# Autodesk Inventor assembly: CarAssembly mk2
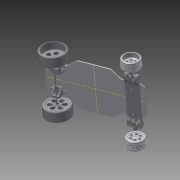
[picture p0: Inventor's stored thumbnail of the model, 180x180]
Saved by Autodesk Inventor 2015 (Build 190159000, 159)
## iProperties
Created: 2014-11-06
Part Number: CarAssembly mk2
Document SubType Name: Assembly
Designer: ah14592
Author: ah14592
## Documents named in this file (10)
- C:\Users\ah14592\Desktop\Inventor\Assembly\CarAssembly mk2.iam
- C:\Users\ah14592\Desktop\Inventor\Steering\Steering Rod\mk1.ipt
- C:\Users\ah14592\Desktop\Inventor\Steering\Steering T\Part3.ipt
- C:\Users\ah14592\Desktop\Inventor\Steering\T Connector Rod\Part1.ipt
- C:\Users\ah14592\Desktop\Inventor\Wheels\Front Wheels\Wheels1.ipt
- C:\Users\ah14592\Desktop\Inventor\Front connectors.ipt
- C:\Users\ah14592\Desktop\Inventor\Base\Basetrimed.ipt
- C:\Users\ah14592\Desktop\Inventor\Rear Axel Holder\holder1_MIR1.ipt
- C:\Users\ah14592\Desktop\Inventor\RearAxel.ipt
- C:\Users\ah14592\Desktop\Inventor\Wheels\Rear Wheels\Wheels1.ipt
## Components (14 placed, 8 different names)
1. mk1:1
2. mk1:2
3. Part3:1
4. Part3:2
5. Part1:1
6. Wheels1:1
7. Wheels1:2
8. Front connectors:1
9. Basetrimed:1
10. holder1_MIR1:1
11. holder1_MIR1:2
12. RearAxel:1
13. Wheels1:3
14. Wheels1:4
## Relationships (30: Mate 20, Flush 10)
- [Mate]: Part3:1 ↔ Part1:1
- [Mate]: Part3:1 ↔ Part1:1
- [Mate]: Part3:2 ↔ Part1:1
- [Mate]: Part3:2 ↔ Part1:1
- [Mate]: mk1:2 ↔ Part3:1
- [Mate]: mk1:2 ↔ Part3:1
- [Mate]: mk1:1 ↔ Part3:1
- [Mate]: mk1:1 ↔ Part3:1
- [Mate]: mk1:1 ↔ Part3:2
- [Mate]: mk1:2 ↔ Part3:2
- [Mate]: Part3:1 ↔ Front connectors:1
- [Mate]: Part3:1 ↔ Front connectors:1
- [Mate]: Wheels1:1 ↔ Front connectors:1
- [Flush] (5 mm): Wheels1:1 ↔ Front connectors:1
- [Mate]: Part1:1 ↔ Basetrimed:1
- [Flush] (30 mm): Part1:1 ↔ Basetrimed:1
- [Mate]: Basetrimed:1 ↔ holder1_MIR1:1
- [Mate]: Basetrimed:1 ↔ holder1_MIR1:2
- [Flush] (5 mm): Basetrimed:1 ↔ holder1_MIR1:1
- [Flush] (5 mm): Basetrimed:1 ↔ holder1_MIR1:2
- [Flush] (15 mm): Basetrimed:1 ↔ holder1_MIR1:2
- [Flush] (15 mm): Basetrimed:1 ↔ holder1_MIR1:1
- [Mate]: holder1_MIR1:2 ↔ RearAxel:1
- [Mate]: holder1_MIR1:1 ↔ RearAxel:1
- [Flush] (34 mm): holder1_MIR1:1 ↔ RearAxel:1
- [Mate]: RearAxel:1 ↔ Wheels1:4
- [Mate]: RearAxel:1 ↔ Wheels1:3
- [Flush] (5 mm): RearAxel:1 ↔ Wheels1:3
- [Flush] (5 mm): RearAxel:1 ↔ Wheels1:4
- [Flush] (28 mm): Part1:1 ↔ Basetrimed:1
## Named parameters: d16_d28 = 0 mm, d17_d29 = 0 mm
